# Autodesk Inventor assembly: Rotado
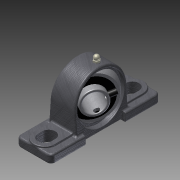
[picture p0: Inventor's stored thumbnail of the model, 180x180]
Saved by Autodesk Inventor 2012 (Build 160160000, 160)
## iProperties
Created: 2014-05-17
Part Number: Rotado
Document SubType Name: Assembly
Designer: Luis
Author: Luis
## Documents named in this file (6)
- E:\3D\Partes en 3D\YO\Chumacera\Rotado.iam
- E:\3D\Partes en 3D\YO\Chumacera\1Rotable.ipt
- E:\3D\Partes en 3D\YO\Chumacera\2Rotable.ipt
- E:\3D\Partes en 3D\YO\Chumacera\3.ipt
- E:\3D\Partes en 3D\YO\Chumacera\4.ipt
- E:\3D\Partes en 3D\YO\Chumacera\5.ipt
## Components (5 placed, 5 different names)
1. 1Rotable:1 — Mate:1, Mate:2, Mate:3, Mate:5
2. 2Rotable:1 — Mate:1, Mate:2, Mate:3, Insert:1, Mate:4
3. 3:1 — Insert:1
4. 4:1 — Mate:4
5. 5:1 — Mate:5
## Relationships (6: Mate 5, Insert 1)
- Mate:1: 1Rotable:1 ↔ 2Rotable:1
- Mate:2: 1Rotable:1 ↔ 2Rotable:1
- Mate:3: 1Rotable:1 ↔ 2Rotable:1
- Insert:1: 2Rotable:1 ↔ 3:1
- Mate:4: 2Rotable:1 ↔ 4:1
- Mate:5: 1Rotable:1 ↔ 5:1
